# Autodesk Inventor assembly: engine
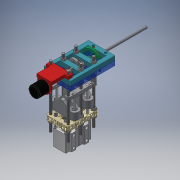
[picture p0: Inventor's stored thumbnail of the model, 180x180]
Saved by Autodesk Inventor 2016 (Build 200138000, 138)
## iProperties
Created: 2017-06-14
Part Number: engine
Document SubType Name: Assembly
Designer: RMcComber
Author: RMcComber
## Documents named in this file (35)
- C:\Users\zimirken\Documents\Steam Engines\two cylinder shaft drive 2\engine.iam
- C:\Users\zimirken\Documents\Steam Engines\two cylinder shaft drive 2\steam cylinder 1.iam
- C:\Users\zimirken\Documents\Steam Engines\two cylinder shaft drive 2\con rod.ipt
- C:\Users\zimirken\Documents\Steam Engines\two cylinder shaft drive 2\engine\Design Accelerator\Bearing1.iam
- C:\Users\zimirken\Documents\Steam Engines\two cylinder shaft drive 2\engine\Design Accelerator\Bearing2.iam
- C:\Users\zimirken\Documents\Steam Engines\two cylinder shaft drive 2\crank web.ipt
- C:\Users\zimirken\Documents\Steam Engines\two cylinder shaft drive 2\frame 1.ipt
- C:\Users\zimirken\Documents\Steam Engines\two cylinder shaft drive 2\cylinder frame.ipt
- C:\Users\zimirken\Documents\Steam Engines\two cylinder shaft drive 2\rotary encoder.ipt
- C:\Users\zimirken\Documents\Steam Engines\two cylinder shaft drive 2\encoder bracket.ipt
- C:\Users\zimirken\Documents\Steam Engines\two cylinder shaft drive 2\sensor.iam
- C:\Users\zimirken\Documents\Steam Engines\two cylinder shaft drive 2\sensor wheel.ipt
- C:\Users\zimirken\Documents\Steam Engines\two cylinder shaft drive 2\sensor bracket coupler.ipt
- C:\Users\zimirken\Documents\Steam Engines\two cylinder shaft drive 2\engine\Design Accelerator\Bearing3.iam
- C:\Users\zimirken\Documents\Steam Engines\two cylinder shaft drive 2\6x8 shaft coupler.ipt
- C:\Users\zimirken\Documents\Steam Engines\two cylinder shaft drive 2\engine\Design Accelerator\Shaft1.iam
- C:\Users\zimirken\Documents\Steam Engines\two cylinder shaft drive 2\engine\Design Accelerator\Shaft2.iam
- C:\Users\zimirken\Documents\Steam Engines\two cylinder shaft drive 2\engine\Design Accelerator\Shaft3.iam
- C:\Users\zimirken\Documents\Steam Engines\two cylinder shaft drive 2\engine\Design Accelerator\Shaft4.iam
- C:\Users\zimirken\Documents\Steam Engines\two cylinder shaft drive 2\engine\Design Accelerator\Shaft5.iam
- C:\Users\zimirken\Documents\Steam Engines\two cylinder shaft drive 2\engine\Design Accelerator\Bearing4.iam
- C:\Users\zimirken\Documents\Steam Engines\two cylinder shaft drive 2\engine\Design Accelerator\Bolted Connection1.iam
- C:\Users\zimirken\Documents\Steam Engines\two cylinder shaft drive 2\engine\Design Accelerator\Bolted Connection2.iam
- C:\Users\zimirken\Documents\Steam Engines\two cylinder shaft drive 2\engine\Design Accelerator\Bolted Connection3.iam
- C:\Users\zimirken\Documents\Steam Engines\two cylinder shaft drive 2\engine\Design Accelerator\Bolted Connection4.iam
- C:\Users\zimirken\Documents\Steam Engines\two cylinder shaft drive 2\frame rod 1.ipt
- C:\Users\zimirken\Documents\Steam Engines\two cylinder shaft drive 2\engine\Design Accelerator\Bolted Connection5.iam
- C:\Users\zimirken\Documents\Inventor\Content Center Files\R2016\en-US\ISO 4032(2)\ISO 4032 - M8 - ISO.ipt
- C:\Users\zimirken\Documents\Steam Engines\two cylinder shaft drive 2\engine\Design Accelerator\Bolted Connection6.iam
- C:\Users\zimirken\Documents\Steam Engines\two cylinder shaft drive 2\engine\Design Accelerator\Bolted Connection7.iam
- C:\Users\zimirken\Documents\Steam Engines\two cylinder shaft drive 2\engine\Design Accelerator\Bolted Connection8.iam
- C:\Users\zimirken\Documents\Steam Engines\two cylinder shaft drive 2\guide rod mount.ipt
- C:\Users\zimirken\Documents\Steam Engines\two cylinder shaft drive 2\guide rod.ipt
- C:\Users\zimirken\Documents\Steam Engines\two cylinder shaft drive 2\combo cross head.ipt
- C:\Users\zimirken\Documents\Steam Engines\two cylinder shaft drive 2\reed switch holder.ipt
## Components (94 placed, 20 different names)
1. steam cylinder 1:1 [sub-assembly] — Mate:1, Flush:1, Flush:2, Mate:32, Mate:236, Mate:239
2. steam cylinder 1:2 [sub-assembly] — Mate:1, Flush:1, Flush:2, Mate:27, Mate:30, Mate:31, Mate:231, Mate:233, Mate:235
3. con rod:1 — Flush:4, Mate:13, Mate:16, Mate:18, Flush:47, Flush:55, Mate:230, Mate:234
4. con rod:2 — Mate:12, Mate:21, Mate:23, Mate:40, Flush:46, Flush:48, Mate:109, Mate:238
5. Bearing:1 [sub-assembly] — Flush:47, Mate:230
6. Bearing:2 [sub-assembly] — Mate:22, Mate:24, Mate:40, Flush:48, Mate:109
7. Bearing:1 [sub-assembly] — Flush:4, Mate:13, Mate:17, Mate:19
8. Bearing:1 [sub-assembly] — Mate:12, Flush:46
9. crank web:1 — Mate:16, Mate:17, Mate:20, Mate:26, Angle:3, Mate:67, Mate:88, Mate:89, Mate:212, Mate:213
10. crank web:2 — Mate:18, Mate:19, Mate:20, Mate:83, Mate:86, Mate:87, Mate:214, Mate:215
11. crank web:3 — Mate:23, Mate:24, Mate:25, Mate:26, Angle:3, Mate:29, Mate:66, Mate:90, Mate:91, Mate:208, Mate:209
12. crank web:4 — Mate:21, Mate:22, Mate:25, Angle:11, Mate:92, Mate:93, Angle:12, Mate:210, Mate:211
13. frame 1:1 — Mate:27, Mate:29, Mate:33, Mate:34, Mate:62, Mate:63, Mate:64, Mate:65, Mate:66, Mate:67, Mate:68, Angle:7, Mate:84, Mate:85, Angle:8, Angle:9, Angle:10, Mate:94, Mate:95, Mate:96, Mate:97, Mate:98, Mate:99, Flush:56, Mate:100, Mate:102, Mate:134, Mate:135, Mate:136, Mate:137, Mate:190, Mate:192, Mate:194, Mate:196, Mate:251
14. cylinder frame:1 — Mate:30, Mate:31, Mate:32, Mate:33, Mate:34, Mate:138, Mate:139, Mate:140, Mate:141, Mate:142, Mate:143, Mate:144, Mate:145, Mate:146, Mate:147, Mate:148, Mate:149, Mate:150, Mate:151, Mate:152, Mate:153, Mate:168, Mate:170, Mate:171, Mate:176, Mate:178, Mate:180, Mate:182, Mate:184, Mate:198, Mate:200, Mate:202, Mate:245, Mate:246, Mate:247, Mate:248, Flush:68, Flush:69, Flush:70, Flush:71
15. frame 1:2 — Mate:62, Mate:63, Mate:64, Mate:70, Mate:71, Flush:58, Mate:154, Flush:59, Flush:60, Mate:155, Mate:156, Flush:61, Mate:157, Mate:160, Mate:162, Mate:164, Mate:166
16. rotary encoder:1 — Mate:38, Mate:39, Mate:69, Mate:81, Mate:82
17. encoder bracket:1 — Mate:38, Mate:39, Mate:68, Mate:69, Mate:70, Mate:71, Flush:62, Flush:63, Mate:158, Mate:159
18. sensor:1 [sub-assembly]
19. sensor wheel:1 — Mate:58, Angle:6, Mate:59, Mate:60, Mate:61, Mate:65, Angle:11
20. sensor bracket coupler:1 — Mate:58, Angle:6, Mate:59, Mate:60, Mate:61, Mate:206, Mate:207, Mate:216, Mate:217
21. Bearing:3 [sub-assembly]
22. 6x8 shaft coupler:1 — Mate:81, Mate:82
23. Shaft:1 [sub-assembly] — Mate:83, Flush:55, Angle:7
24. Bearing:1 [sub-assembly] — Mate:84, Mate:85
25. Shaft:2 [sub-assembly] — Mate:86, Mate:87, Angle:8
26. Shaft:3 [sub-assembly] — Mate:88, Mate:89, Angle:9
27. Shaft:4 [sub-assembly] — Mate:90, Mate:91, Angle:10
28. Shaft:5 [sub-assembly] — Mate:92, Mate:93, Angle:12
29. Bearing:1 [sub-assembly] — Mate:94, Mate:95
30. Bearing:1 [sub-assembly] — Mate:96, Mate:97
31. Bearing:1 [sub-assembly] — Mate:98, Mate:99
32. Bearing:4 [sub-assembly] — Flush:56, Mate:100, Mate:101
33. Bearing:6 [sub-assembly] — Mate:101, Mate:102
34. Bearing:9 [sub-assembly]
35. Bolted Connection:1 [sub-assembly]
36. Bolted Connection:2 [sub-assembly]
37. Bolted Connection:3 [sub-assembly]
38. Bolted Connection:4 [sub-assembly]
39. Bolted Connection:5 [sub-assembly]
40. Bolted Connection:6 [sub-assembly]
41. Bolted Connection:7 [sub-assembly]
42. Bolted Connection:8 [sub-assembly]
43. Bolted Connection:9 [sub-assembly]
44. Bolted Connection:10 [sub-assembly]
45. Bolted Connection:11 [sub-assembly] — Mate:134, Mate:135
46. Bolted Connection:12 [sub-assembly] — Mate:136, Mate:137
47. frame rod 1:1 — Flush:60, Mate:156, Mate:165, Mate:179, Mate:181, Mate:244, Mate:250
48. frame rod 1:2 — Flush:59, Mate:155, Mate:163, Mate:197, Mate:201
49. frame rod 1:3 — Flush:58, Mate:154, Mate:161, Mate:169, Mate:199, Mate:226, Mate:249
50. frame rod 1:4 — Flush:61, Mate:157, Mate:167, Mate:177, Mate:183, Mate:191
51. frame rod 1:5 — Flush:62, Mate:159, Mate:185, Mate:193, Mate:243
52. frame rod 1:6 — Flush:63, Mate:158, Mate:195, Mate:203, Mate:225
53. Bolted Connection:13 [sub-assembly] — Mate:138, Mate:139
54. Bolted Connection:14 [sub-assembly] — Mate:146, Mate:147
55. Bolted Connection:15 [sub-assembly] — Mate:148, Mate:149
56. Bolted Connection:16 [sub-assembly] — Mate:142, Mate:143
57. Bolted Connection:17 [sub-assembly] — Mate:140, Mate:141
58. Bolted Connection:18 [sub-assembly] — Mate:144, Mate:145
59. Bolted Connection:19 [sub-assembly] — Mate:152, Mate:153
60. Bolted Connection:20 [sub-assembly] — Mate:150, Mate:151
61. ISO 4032 M8:1 — Mate:160, Mate:161
62. ISO 4032 M8:2 — Mate:162, Mate:163
63. ISO 4032 M8:3 — Mate:164, Mate:165
64. ISO 4032 M8:4 — Mate:180, Mate:181
65. ISO 4032 M8:5 — Mate:190, Mate:191
66. ISO 4032 M8:6 — Mate:176, Mate:177
67. ISO 4032 M8:7 — Mate:168, Mate:169
68. ISO 4032 M8:8 — Mate:166, Mate:167
69. ISO 4032 M8:9 — Mate:200, Mate:201
70. ISO 4032 M8:10 — Mate:192, Mate:193
71. ISO 4032 M8:11 — Mate:198, Mate:199
72. ISO 4032 M8:12 — Mate:184, Mate:185
73. ISO 4032 M8:14 — Mate:178, Mate:179
74. ISO 4032 M8:16 — Mate:170, Mate:171
75. ISO 4032 M8:18 — Mate:194, Mate:195
76. ISO 4032 M8:20 — Mate:196, Mate:197
77. ISO 4032 M8:21 — Mate:182, Mate:183
78. ISO 4032 M8:22 — Mate:202, Mate:203
79. Bolted Connection:21 [sub-assembly]
80. Bolted Connection:22 [sub-assembly] — Mate:206, Mate:207
81. Bolted Connection:23 [sub-assembly] — Mate:208, Mate:209
82. Bolted Connection:24 [sub-assembly] — Mate:210, Mate:211
83. Bolted Connection:25 [sub-assembly] — Mate:212, Mate:213
84. Bolted Connection:26 [sub-assembly] — Mate:214, Mate:215
85. Bolted Connection:27 [sub-assembly] — Mate:216, Mate:217
86. guide rod mount:2 — Mate:225, Mate:226, Flush:64, Flush:65
87. guide rod:1 — Flush:64, Mate:237, Mate:247, Flush:68
88. guide rod:2 — Flush:65, Mate:232, Mate:248, Flush:69
89. combo cross head:1 — Mate:231, Mate:232, Mate:233, Mate:234, Mate:235
90. combo cross head:2 — Mate:236, Mate:237, Mate:238, Mate:239
91. guide rod mount:4 — Mate:243, Mate:244, Flush:66, Flush:67
92. guide rod:3 — Flush:67, Mate:246, Flush:70
93. guide rod:4 — Flush:66, Mate:245, Flush:71
94. reed switch holder:1 — Mate:249, Mate:250, Mate:251
## Relationships (186: Mate 156, Flush 22, Angle 8)
- Mate:1: steam cylinder 1:1 ↔ steam cylinder 1:2
- Flush:1: steam cylinder 1:1 ↔ steam cylinder 1:2
- Flush:2: steam cylinder 1:1 ↔ steam cylinder 1:2
- Mate:12: con rod:2 ↔ Bearing:1
- Flush:4: con rod:1 ↔ Bearing:1
- Mate:13: con rod:1 ↔ Bearing:1
- Mate:16: con rod:1 ↔ crank web:1
- Mate:17: Bearing:1 ↔ crank web:1
- Mate:18: con rod:1 ↔ crank web:2
- Mate:19: Bearing:1 ↔ crank web:2
- Mate:20: crank web:1 ↔ crank web:2
- Mate:21: con rod:2 ↔ crank web:4
- Mate:22: Bearing:2 ↔ crank web:4
- Mate:23: con rod:2 ↔ crank web:3
- Mate:24: Bearing:2 ↔ crank web:3
- Mate:25: crank web:3 ↔ crank web:4
- Mate:26: crank web:1 ↔ crank web:3
- Angle:3 (-90 deg): crank web:1 ↔ crank web:3
- Mate:27 (144 mm): steam cylinder 1:2 ↔ frame 1:1
- Mate:29: crank web:3 ↔ frame 1:1
- Mate:30 (20 mm): steam cylinder 1:2 ↔ cylinder frame:1
- Mate:31: steam cylinder 1:2 ↔ cylinder frame:1
- Mate:32: steam cylinder 1:1 ↔ cylinder frame:1
- Mate:33: frame 1:1 ↔ cylinder frame:1
- Mate:34: frame 1:1 ↔ cylinder frame:1
- Mate:38: rotary encoder:1 ↔ encoder bracket:1
- Mate:39: rotary encoder:1 ↔ encoder bracket:1
- Mate:40: con rod:2 ↔ Bearing:2
- Flush:47: con rod:1 ↔ Bearing:1
- Flush:46: con rod:2 ↔ Bearing:1
- Flush:48: con rod:2 ↔ Bearing:2
- Mate:58: sensor wheel:1 ↔ sensor bracket coupler:1
- Angle:6 (180 deg): sensor wheel:1 ↔ sensor bracket coupler:1
- Mate:59 (1 mm): sensor wheel:1 ↔ sensor bracket coupler:1
- Mate:60: sensor wheel:1 ↔ sensor bracket coupler:1
- Mate:61: sensor wheel:1 ↔ sensor bracket coupler:1
- Mate:62: frame 1:1 ↔ frame 1:2
- Mate:63: frame 1:1 ↔ frame 1:2
- Mate:64: frame 1:1 ↔ frame 1:2
- Mate:65: frame 1:1 ↔ sensor wheel:1
- Mate:66: crank web:3 ↔ frame 1:1
- Mate:67: crank web:1 ↔ frame 1:1
- Mate:68: frame 1:1 ↔ encoder bracket:1
- Mate:69: rotary encoder:1 ↔ encoder bracket:1
- Mate:70: frame 1:2 ↔ encoder bracket:1
- Mate:71: frame 1:2 ↔ encoder bracket:1
- Mate:81 (5 mm): rotary encoder:1 ↔ 6x8 shaft coupler:1
- Mate:82: rotary encoder:1 ↔ 6x8 shaft coupler:1
- Mate:83: crank web:2 ↔ Shaft:1
- Flush:55: con rod:1 ↔ Shaft:1
- Angle:7 (0 deg): frame 1:1 ↔ Shaft:1
- Mate:84: frame 1:1 ↔ Bearing:1
- Mate:85: frame 1:1 ↔ Bearing:1
- Mate:86: crank web:2 ↔ Shaft:2
- Mate:87: crank web:2 ↔ Shaft:2
- Angle:8 (0 deg): frame 1:1 ↔ Shaft:2
- Mate:88: crank web:1 ↔ Shaft:3
- Mate:89: crank web:1 ↔ Shaft:3
- Angle:9 (0 deg): frame 1:1 ↔ Shaft:3
- Mate:90: crank web:3 ↔ Shaft:4
- Mate:91: crank web:3 ↔ Shaft:4
- Angle:10 (0 deg): frame 1:1 ↔ Shaft:4
- Angle:11 (0 deg): crank web:4 ↔ sensor wheel:1
- Mate:92: crank web:4 ↔ Shaft:5
- Mate:93: crank web:4 ↔ Shaft:5
- Angle:12 (0 deg): crank web:4 ↔ Shaft:5
- Mate:94: frame 1:1 ↔ Bearing:1
- Mate:95: frame 1:1 ↔ Bearing:1
- Mate:96: frame 1:1 ↔ Bearing:1
- Mate:97: frame 1:1 ↔ Bearing:1
- Mate:98: frame 1:1 ↔ Bearing:1
- Mate:99: frame 1:1 ↔ Bearing:1
- Flush:56: frame 1:1 ↔ Bearing:4
- Mate:100: frame 1:1 ↔ Bearing:4
- Mate:101: Bearing:4 ↔ Bearing:6
- Mate:102: frame 1:1 ↔ Bearing:6
- Mate:109: con rod:2 ↔ Bearing:2
- Mate:134: frame 1:1 ↔ Bolted Connection:11
- Mate:135: frame 1:1 ↔ Bolted Connection:11
- Mate:136: frame 1:1 ↔ Bolted Connection:12
- Mate:137: frame 1:1 ↔ Bolted Connection:12
- Mate:138: cylinder frame:1 ↔ Bolted Connection:13
- Mate:139: cylinder frame:1 ↔ Bolted Connection:13
- Mate:140: cylinder frame:1 ↔ Bolted Connection:17
- Mate:141: cylinder frame:1 ↔ Bolted Connection:17
- Mate:142: cylinder frame:1 ↔ Bolted Connection:16
- Mate:143: cylinder frame:1 ↔ Bolted Connection:16
- Mate:144: cylinder frame:1 ↔ Bolted Connection:18
- Mate:145: cylinder frame:1 ↔ Bolted Connection:18
- Mate:146: cylinder frame:1 ↔ Bolted Connection:14
- Mate:147: cylinder frame:1 ↔ Bolted Connection:14
- Mate:148: cylinder frame:1 ↔ Bolted Connection:15
- Mate:149: cylinder frame:1 ↔ Bolted Connection:15
- Mate:150: cylinder frame:1 ↔ Bolted Connection:20
- Mate:151: cylinder frame:1 ↔ Bolted Connection:20
- Mate:152: cylinder frame:1 ↔ Bolted Connection:19
- Mate:153: cylinder frame:1 ↔ Bolted Connection:19
- Flush:58 (-20 mm): frame 1:2 ↔ frame rod 1:3
- Mate:154: frame 1:2 ↔ frame rod 1:3
- Flush:59 (-20 mm): frame 1:2 ↔ frame rod 1:2
- Flush:60 (-20 mm): frame 1:2 ↔ frame rod 1:1
- Mate:155: frame 1:2 ↔ frame rod 1:2
- Mate:156: frame 1:2 ↔ frame rod 1:1
- Flush:61 (-20 mm): frame 1:2 ↔ frame rod 1:4
- Mate:157: frame 1:2 ↔ frame rod 1:4
- Flush:62 (-10 mm): encoder bracket:1 ↔ frame rod 1:5
- Flush:63 (-10 mm): encoder bracket:1 ↔ frame rod 1:6
- Mate:158: encoder bracket:1 ↔ frame rod 1:6
- Mate:159: encoder bracket:1 ↔ frame rod 1:5
- Mate:160: frame 1:2 ↔ ISO 4032 M8:1
- Mate:161: frame rod 1:3 ↔ ISO 4032 M8:1
- Mate:162: frame 1:2 ↔ ISO 4032 M8:2
- Mate:163: frame rod 1:2 ↔ ISO 4032 M8:2
- Mate:164: frame 1:2 ↔ ISO 4032 M8:3
- Mate:165: frame rod 1:1 ↔ ISO 4032 M8:3
- Mate:166: frame 1:2 ↔ ISO 4032 M8:8
- Mate:167: frame rod 1:4 ↔ ISO 4032 M8:8
- Mate:168: cylinder frame:1 ↔ ISO 4032 M8:7
- Mate:169: frame rod 1:3 ↔ ISO 4032 M8:7
- Mate:170: cylinder frame:1 ↔ ISO 4032 M8:16
- Mate:171: cylinder frame:1 ↔ ISO 4032 M8:16
- Mate:176: cylinder frame:1 ↔ ISO 4032 M8:6
- Mate:177: frame rod 1:4 ↔ ISO 4032 M8:6
- Mate:178: cylinder frame:1 ↔ ISO 4032 M8:14
- Mate:179: frame rod 1:1 ↔ ISO 4032 M8:14
- Mate:180: cylinder frame:1 ↔ ISO 4032 M8:4
- Mate:181: frame rod 1:1 ↔ ISO 4032 M8:4
- Mate:182: cylinder frame:1 ↔ ISO 4032 M8:21
- Mate:183: frame rod 1:4 ↔ ISO 4032 M8:21
- Mate:184: cylinder frame:1 ↔ ISO 4032 M8:12
- Mate:185: frame rod 1:5 ↔ ISO 4032 M8:12
- Mate:190: frame 1:1 ↔ ISO 4032 M8:5
- Mate:191: frame rod 1:4 ↔ ISO 4032 M8:5
- Mate:192: frame 1:1 ↔ ISO 4032 M8:10
- Mate:193: frame rod 1:5 ↔ ISO 4032 M8:10
- Mate:194: frame 1:1 ↔ ISO 4032 M8:18
- Mate:195: frame rod 1:6 ↔ ISO 4032 M8:18
- Mate:196: frame 1:1 ↔ ISO 4032 M8:20
- Mate:197: frame rod 1:2 ↔ ISO 4032 M8:20
- Mate:198: cylinder frame:1 ↔ ISO 4032 M8:11
- Mate:199: frame rod 1:3 ↔ ISO 4032 M8:11
- Mate:200: cylinder frame:1 ↔ ISO 4032 M8:9
- Mate:201: frame rod 1:2 ↔ ISO 4032 M8:9
- Mate:202: cylinder frame:1 ↔ ISO 4032 M8:22
- Mate:203: frame rod 1:6 ↔ ISO 4032 M8:22
- Mate:206: sensor bracket coupler:1 ↔ Bolted Connection:22
- Mate:207: sensor bracket coupler:1 ↔ Bolted Connection:22
- Mate:208: crank web:3 ↔ Bolted Connection:23
- Mate:209: crank web:3 ↔ Bolted Connection:23
- Mate:210: crank web:4 ↔ Bolted Connection:24
- Mate:211: crank web:4 ↔ Bolted Connection:24
- Mate:212: crank web:1 ↔ Bolted Connection:25
- Mate:213: crank web:1 ↔ Bolted Connection:25
- Mate:214: crank web:2 ↔ Bolted Connection:26
- Mate:215: crank web:2 ↔ Bolted Connection:26
- Mate:216: sensor bracket coupler:1 ↔ Bolted Connection:27
- Mate:217: sensor bracket coupler:1 ↔ Bolted Connection:27
- Mate:225: frame rod 1:6 ↔ guide rod mount:2
- Mate:226: frame rod 1:3 ↔ guide rod mount:2
- Flush:64: guide rod mount:2 ↔ guide rod:1
- Flush:65: guide rod mount:2 ↔ guide rod:2
- Mate:230: con rod:1 ↔ Bearing:1
- Mate:231: steam cylinder 1:2 ↔ combo cross head:1
- Mate:232: guide rod:2 ↔ combo cross head:1
- Mate:233: steam cylinder 1:2 ↔ combo cross head:1
- Mate:234: con rod:1 ↔ combo cross head:1
- Mate:235 (38 mm): steam cylinder 1:2 ↔ combo cross head:1
- Mate:236: steam cylinder 1:1 ↔ combo cross head:2
- Mate:237: guide rod:1 ↔ combo cross head:2
- Mate:238: con rod:2 ↔ combo cross head:2
- Mate:239 (38 mm): steam cylinder 1:1 ↔ combo cross head:2
- Mate:243: frame rod 1:5 ↔ guide rod mount:4
- Mate:244: frame rod 1:1 ↔ guide rod mount:4
- Flush:66: guide rod mount:4 ↔ guide rod:4
- Flush:67: guide rod mount:4 ↔ guide rod:3
- Mate:245: cylinder frame:1 ↔ guide rod:4
- Mate:246: cylinder frame:1 ↔ guide rod:3
- Mate:247: cylinder frame:1 ↔ guide rod:1
- Mate:248: cylinder frame:1 ↔ guide rod:2
- Flush:68: cylinder frame:1 ↔ guide rod:1
- Flush:69: cylinder frame:1 ↔ guide rod:2
- Flush:70: cylinder frame:1 ↔ guide rod:3
- Flush:71: cylinder frame:1 ↔ guide rod:4
- Mate:249: frame rod 1:3 ↔ reed switch holder:1
- Mate:250: frame rod 1:1 ↔ reed switch holder:1
- Mate:251: frame 1:1 ↔ reed switch holder:1
